# Autodesk Inventor assembly: Rear_Frame_Fixer
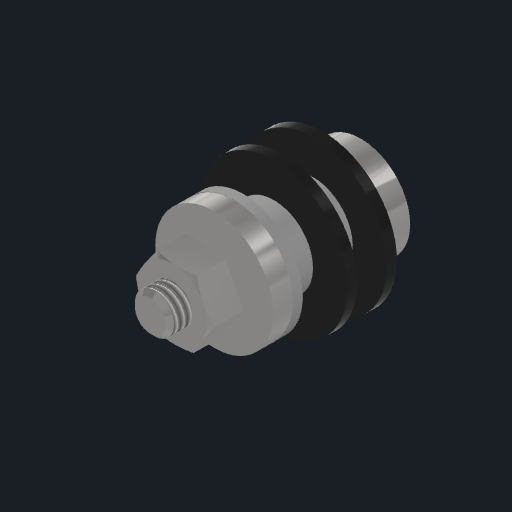
[picture p0: Inventor's stored thumbnail of the model, 512x512]
Saved by Autodesk Inventor 2024.3 (Build 283343000, 343)
## iProperties
Created: 2024-01-28
Part Number: Rear_Frame_Fixer
Document SubType Name: Assembly
Designer: 김대겸
Author: 김대겸
## Documents named in this file (7)
- C:\Users\ASUS\Desktop\test\v3_Frame\Rear_Frame_Fixer.iam
- C:\Users\ASUS\Desktop\test\v1_Frame\MISUMI\C-WSSA12-4-2.ipt
- C:\Users\ASUS\Desktop\test\v3_Frame\MISUMI\NBW-0815-10.ipt
- C:\Users\ASUS\Desktop\test\v1_Frame\MISUMI\SLBNR4.ipt
- C:\Users\ASUS\Desktop\test\v3_Frame\MISUMI\DBB4-10-8.ipt
- C:\Users\ASUS\Desktop\test\v2_Frame\MISUMI\80F-0608.ipt
- C:\Users\ASUS\Desktop\test\v3_Frame\MISUMI\NBW-0612-10.ipt
## Components (7 placed, 6 different names)
1. C-WSSA12-4-2:1 — 삽입:2, 삽입:3, 삽입:4
2. NBW-0815-10:1 — 삽입:5
3. SLBNR4:1 — 삽입:3, 각도:1
4. DBB4-10-8:1 — 삽입:2, 각도:1, 삽입:6
5. 80F-0608:1 — 삽입:4, 삽입:5
6. NBW-0612-10:1 — 삽입:6, 삽입:7
7. NBW-0815-10:2 — 삽입:7
## Relationships (7: Insert 6, Angle 1)
- 삽입:2 [Insert]: C-WSSA12-4-2:1 ↔ DBB4-10-8:1
- 삽입:3 [Insert] (1 mm): C-WSSA12-4-2:1 ↔ SLBNR4:1
- 각도:1 [Angle] (0 deg): SLBNR4:1 ↔ DBB4-10-8:1
- 삽입:4 [Insert]: C-WSSA12-4-2:1 ↔ 80F-0608:1
- 삽입:5 [Insert] (3 mm): NBW-0815-10:1 ↔ 80F-0608:1
- 삽입:6 [Insert]: DBB4-10-8:1 ↔ NBW-0612-10:1
- 삽입:7 [Insert]: NBW-0612-10:1 ↔ NBW-0815-10:2
